# Autodesk Inventor assembly: RoadBot Electronics Module - with Jack - r3
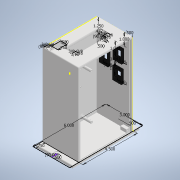
[picture p0: Inventor's stored thumbnail of the model, 180x180]
Saved by Autodesk Inventor 2020 (Build 240168000, 168)
## iProperties
Created: 2022-03-31
Part Number: RoadBot Electronics Module - with Jack - r3
Document SubType Name: Assembly
Designer: Beaucage
Author: Beaucage
## Documents named in this file (3)
- V:\AFL\Drawings\RoadBot Electronics Module - with Jack - r3.iam
- V:\AFL\Drawings\Keystone_Jack_Single_Receptacle (1).ipt
- V:\AFL\Drawings\Compute Module for RoadBot Rail-r2.ipt
## Components (4 placed, 2 different names)
1. Compute Module for RoadBot Rail-r2:1 — Mate:1, Mate:2, Flush:1, Mate:3, Mate:4, Flush:2, Mate:5, Flush:3, Mate:6
2. Keystone_Jack_Single_Receptacle (1):1 — Mate:1, Mate:2, Flush:1
3. Keystone_Jack_Single_Receptacle (1):2 — Mate:3, Mate:4, Flush:2
4. Keystone_Jack_Single_Receptacle (1):3 — Mate:5, Flush:3, Mate:6
## Relationships (9: Mate 6, Flush 3)
- Mate:1: Compute Module for RoadBot Rail-r2:1 ↔ Keystone_Jack_Single_Receptacle (1):1
- Mate:2: Compute Module for RoadBot Rail-r2:1 ↔ Keystone_Jack_Single_Receptacle (1):1
- Flush:1: Compute Module for RoadBot Rail-r2:1 ↔ Keystone_Jack_Single_Receptacle (1):1
- Mate:3: Compute Module for RoadBot Rail-r2:1 ↔ Keystone_Jack_Single_Receptacle (1):2
- Mate:4: Compute Module for RoadBot Rail-r2:1 ↔ Keystone_Jack_Single_Receptacle (1):2
- Flush:2: Compute Module for RoadBot Rail-r2:1 ↔ Keystone_Jack_Single_Receptacle (1):2
- Mate:5: Compute Module for RoadBot Rail-r2:1 ↔ Keystone_Jack_Single_Receptacle (1):3
- Flush:3: Compute Module for RoadBot Rail-r2:1 ↔ Keystone_Jack_Single_Receptacle (1):3
- Mate:6: Compute Module for RoadBot Rail-r2:1 ↔ Keystone_Jack_Single_Receptacle (1):3
